# Autodesk Inventor assembly: plate_assembly_stacked
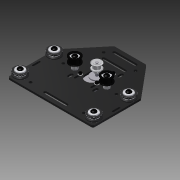
[picture p0: Inventor's stored thumbnail of the model, 180x180]
Saved by Autodesk Inventor 2014 (Build 180170000, 170)
## iProperties
Created: 2013-05-29
Part Number: plate_assembly_stacked
Document SubType Name: Assembly
Designer: Edward
Mass: 864.739 g
Surface Area: 894.967 cm^2
Volume: 163.574 cm^3
Density: 5.28654 g/cm^3
Author: Edward
## Documents named in this file (14)
- C:\Users\Edward\Desktop\Shapeoko_v2.0\plate_assembly_stacked.iam
- C:\Users\Edward\Desktop\Shapeoko_v2.0\S2_mm.ipt
- C:\Users\Edward\Desktop\Shapeoko_v2.0\B18033.ipt
- C:\Users\Edward\Desktop\Shapeoko_v2.0\B30037.iam
- C:\Users\Edward\Desktop\Shapeoko_v2.0\91239A233.ipt
- C:\Users\Edward\Desktop\Shapeoko_v2.0\SM-H03.ipt
- C:\Users\Edward\Desktop\Shapeoko_v2.0\SM-H04.ipt
- C:\Users\Edward\Desktop\Shapeoko_v2.0\SM-E01.ipt
- C:\Users\Edward\Desktop\Shapeoko_v2.0\B30041.iam
- C:\Users\Edward\Desktop\Shapeoko_v2.0\91239A236.ipt
- C:\Users\Edward\Desktop\Shapeoko_v2.0\91166A210.ipt
- C:\Users\Edward\Desktop\Shapeoko_v2.0\91290A113.ipt
- C:\Users\Edward\Desktop\Shapeoko_v2.0\a_6a51-020df0606.ipt
- C:\Users\Edward\Desktop\Shapeoko_v2.0\AS38-12-20.ipt
## Components (43 placed, 13 different names)
1. S2_mm:1 — Insert:3, Insert:5, Insert:9, Mate:2, Insert:10, Mate:4, Insert:15, Insert:16, Insert:18, Insert:21, Insert:24, Insert:26
2. B18033:1 — Insert:10, Mate:3
3. B18033:2 — Mate:1, Insert:9
4. B30037:4 [sub-assembly] — Insert:2, Insert:4
5. SM-H03:1 — Insert:2, Insert:3
6. 91239A233:2 — Insert:4
7. SM-H03:2 — Insert:11, Mate:4
8. SM-H04:2 — Insert:6
9. SM-H03:4 — Insert:16, Insert:17
10. SM-H03:5 — Insert:14, Insert:15
11. SM-H03:6 — Insert:7, Mate:2
12. SM-H03:7 — Insert:5, Insert:6
13. 91239A233:3 — Insert:8, Mate:1
14. B30037:5 [sub-assembly] — Insert:7, Insert:8
15. 91239A233:4 — Insert:12, Mate:3
16. B30037:6 [sub-assembly] — Insert:11, Insert:12
17. 91239A233:5 — Insert:13
18. B30037:7 [sub-assembly] — Insert:13, Insert:14
19. SM-H04:3 — Insert:17
20. SM-E01:1 — Insert:18, Insert:32, Insert:36, Insert:37, Insert:38, Mate:5
21. B30041:1 [sub-assembly] — Flush:1
22. B30041:2 [sub-assembly] — Insert:21
23. 91239A236:2
24. SM-H03:8 — Insert:23, Insert:24
25. SM-H04:4 — Insert:23
26. 91239A236:1
27. SM-H04:5 — Insert:27
28. SM-H03:9 — Insert:26, Insert:27
29. AS38-12-20:1 — Insert:39
30. AS38-12-20:2 — Insert:41
31. 91166A210:1 — Insert:31, Insert:32
32. 91290A113:1 — Insert:31
33. 91166A210:2 — Insert:33, Insert:37
34. 91290A113:2 — Insert:33
35. 91166A210:3 — Insert:34, Insert:38
36. 91290A113:3 — Insert:34
37. 91166A210:4 — Insert:35, Insert:36
38. 91290A113:4 — Insert:35
39. a_6a51-020df0606:1 — Mate:5, Flush:1
40. SM-H03:10 — Insert:39, Insert:40
41. SM-H03:11 — Insert:40
42. SM-H03:12 — Insert:42
43. SM-H03:13 — Insert:41, Insert:42
## Relationships (45: Insert 39, Mate 5, Flush 1)
- Insert:2: B30037:4 ↔ SM-H03:1
- Insert:3: S2_mm:1 ↔ SM-H03:1
- Insert:4: B30037:4 ↔ 91239A233:2
- Insert:5: S2_mm:1 ↔ SM-H03:7
- Insert:6: SM-H04:2 ↔ SM-H03:7
- Insert:7: SM-H03:6 ↔ B30037:5
- Insert:8: 91239A233:3 ↔ B30037:5
- Mate:1: B18033:2 ↔ 91239A233:3
- Insert:9: S2_mm:1 ↔ B18033:2
- Mate:2: S2_mm:1 ↔ SM-H03:6
- Insert:10: S2_mm:1 ↔ B18033:1
- Insert:11: SM-H03:2 ↔ B30037:6
- Insert:12: 91239A233:4 ↔ B30037:6
- Mate:3: B18033:1 ↔ 91239A233:4
- Mate:4: S2_mm:1 ↔ SM-H03:2
- Insert:13: 91239A233:5 ↔ B30037:7
- Insert:14: SM-H03:5 ↔ B30037:7
- Insert:15: S2_mm:1 ↔ SM-H03:5
- Insert:16: S2_mm:1 ↔ SM-H03:4
- Insert:17: SM-H03:4 ↔ SM-H04:3
- Insert:18: S2_mm:1 ↔ SM-E01:1
- Insert:21 (9.525 mm): S2_mm:1 ↔ B30041:2
- [Insert]: B30041:1 ↔ 91239A236:2
- Insert:23: SM-H03:8 ↔ SM-H04:4
- Insert:24: S2_mm:1 ↔ SM-H03:8
- [Insert]: B30041:2 ↔ 91239A236:1
- Insert:26: S2_mm:1 ↔ SM-H03:9
- Insert:27: SM-H04:5 ↔ SM-H03:9
- [Insert]: B30041:2 ↔ AS38-12-20:1
- [Insert]: S2_mm:1 ↔ AS38-12-20:2
- [Insert]: B30041:1 ↔ AS38-12-20:2
- Insert:31: 91166A210:1 ↔ 91290A113:1
- Insert:32 (4 mm): SM-E01:1 ↔ 91166A210:1
- Insert:33: 91166A210:2 ↔ 91290A113:2
- Insert:34: 91166A210:3 ↔ 91290A113:3
- Insert:35: 91166A210:4 ↔ 91290A113:4
- Insert:36 (4 mm): SM-E01:1 ↔ 91166A210:4
- Insert:37 (4 mm): SM-E01:1 ↔ 91166A210:2
- Insert:38 (4 mm): SM-E01:1 ↔ 91166A210:3
- Mate:5: SM-E01:1 ↔ a_6a51-020df0606:1
- Flush:1 (0.65 mm): B30041:1 ↔ a_6a51-020df0606:1
- Insert:39: AS38-12-20:1 ↔ SM-H03:10
- Insert:40: SM-H03:10 ↔ SM-H03:11
- Insert:41: AS38-12-20:2 ↔ SM-H03:13
- Insert:42: SM-H03:12 ↔ SM-H03:13
